# Autodesk Inventor assembly: Bottom layer
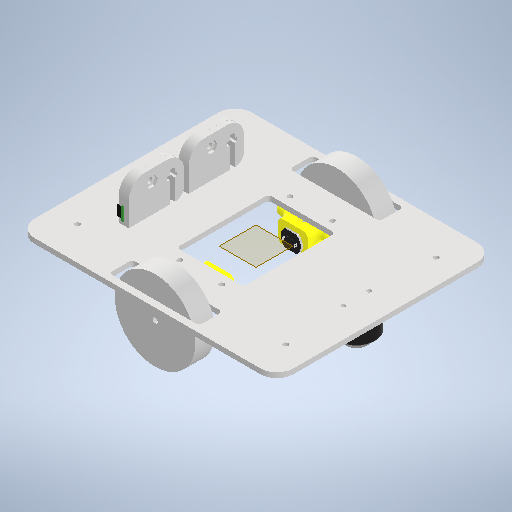
[picture p0: Inventor's stored thumbnail of the model, 512x512]
Saved by Autodesk Inventor 2025.1 (Build 291241000, 241)
## iProperties
Created: 2024-10-04
Part Number: Bottom layer
Document SubType Name: Assembly
Designer: bw1293
Author: bw1293
## Documents named in this file (5)
- C:\Users\benja\OneDrive\Documents\PlatformIO\Projects\241025-214150-nano33ble\GEOFF-2.0\CAD\Bottom layer.iam
- C:\Users\benja\OneDrive\Documents\PlatformIO\Projects\241025-214150-nano33ble\GEOFF-2.0\CAD\Bottom layer2.ipt
- C:\Users\benja\OneDrive\Documents\PlatformIO\Projects\241025-214150-nano33ble\GEOFF-2.0\CAD\Motor assembly.iam
- C:\Users\benja\OneDrive\Documents\PlatformIO\Projects\241025-214150-nano33ble\GEOFF-2.0\CAD\0.75in Ball Caster (Pololu).ipt
- C:\Users\benja\OneDrive\Documents\PlatformIO\Projects\241025-214150-nano33ble\GEOFF-2.0\CAD\IR Sensor Mount.iam
## Components (7 placed, 4 different names)
1. Bottom layer2:1 — Insert:1, Insert:2, Insert:3, Insert:4, Insert:5, Insert:6, Insert:7, Insert:8, Mate:1, Mate:2, Mate:3, Mate:4, Mate:5, Mate:6
2. Motor assembly:1 [sub-assembly] — Insert:3, Insert:4
3. Motor assembly:2 [sub-assembly] — Insert:1, Insert:2
4. 0.75in Ball Caster (Pololu):1 — Insert:5, Insert:6
5. 0.75in Ball Caster (Pololu):2 — Insert:7, Insert:8
6. IR Sensor Mount:1 [sub-assembly] — Mate:4, Mate:5, Mate:6
7. IR Sensor Mount:2 [sub-assembly] — Mate:1, Mate:2, Mate:3
## Relationships (14: Insert 8, Mate 6)
- Insert:1: Bottom layer2:1 ↔ Motor assembly:2
- Insert:2: Bottom layer2:1 ↔ Motor assembly:2
- Insert:3: Bottom layer2:1 ↔ Motor assembly:1
- Insert:4: Bottom layer2:1 ↔ Motor assembly:1
- Insert:5: Bottom layer2:1 ↔ 0.75in Ball Caster (Pololu):1
- Insert:6: Bottom layer2:1 ↔ 0.75in Ball Caster (Pololu):1
- Insert:7: Bottom layer2:1 ↔ 0.75in Ball Caster (Pololu):2
- Insert:8: Bottom layer2:1 ↔ 0.75in Ball Caster (Pololu):2
- Mate:1: Bottom layer2:1 ↔ IR Sensor Mount:2
- Mate:2: Bottom layer2:1 ↔ IR Sensor Mount:2
- Mate:3: Bottom layer2:1 ↔ IR Sensor Mount:2
- Mate:4: Bottom layer2:1 ↔ IR Sensor Mount:1
- Mate:5: Bottom layer2:1 ↔ IR Sensor Mount:1
- Mate:6: Bottom layer2:1 ↔ IR Sensor Mount:1
